# Autodesk Inventor assembly: Functioning elevator (frame 2)
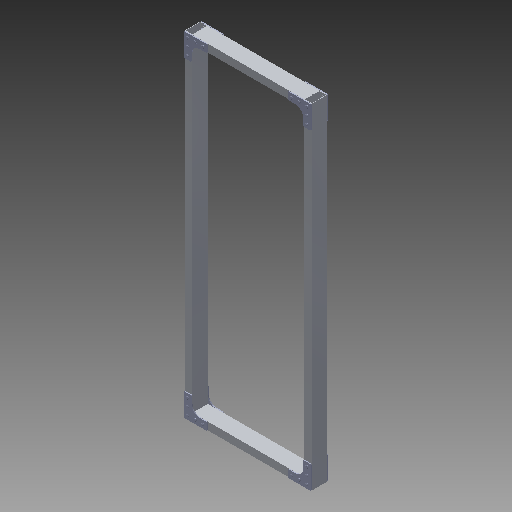
[picture p0: Inventor's stored thumbnail of the model, 512x512]
Saved by Autodesk Inventor 2019 (Build 230136000, 136)
## iProperties
Created: 2019-01-19
Part Number: Functioning elevator (frame 2)
Document SubType Name: Assembly
Designer: josh
Mass: 2087.98 g
Surface Area: 9404.6 cm^2
Volume: 773.327 cm^3
Density: 2.7 g/cm^3
Author: josh
## Documents named in this file (4)
- D:\Synthesis Robots\Epsilon\Epsilon elavator lift\Functioning elevator (frame 2).iam
- D:\Synthesis Robots\Epsilon\Epsilon elavator lift\Functioning elevator parts\Example Fixed Tube.ipt
- D:\Synthesis Robots\Epsilon\Epsilon elavator lift\Functioning elevator parts\am-3860 90 Gusset with Rivets.iam
- D:\Synthesis Robots\Epsilon\Epsilon elavator lift\Functioning elevator parts\Example Cross Frame Tube - Copy.ipt
## Components (12 placed, 3 different names)
1. Example Fixed Tube:1 — Mate:12, Flush:24, Mate:16, Flush:29, Flush:30, Flush:31, Mate:20, Flush:32
2. Example Fixed Tube:2 — Flush:22, Flush:23, Mate:14, Mate:15, Mate:17, Mate:18
3. am-3860 90 Gusset with Rivets:1 [sub-assembly] — Flush:22
4. am-3860 90 Gusset with Rivets:2 [sub-assembly] — Flush:23, Flush:25, Mate:13, Mate:14
5. am-3860 90 Gusset with Rivets:3 [sub-assembly] — Mate:11, Mate:12, Flush:24
6. am-3860 90 Gusset with Rivets:4 [sub-assembly] — Mate:10, Flush:32, Flush:33
7. am-3860 90 Gusset with Rivets:5 [sub-assembly] — Mate:18, Mate:19, Flush:27
8. am-3860 90 Gusset with Rivets:6 [sub-assembly] — Flush:26
9. am-3860 90 Gusset with Rivets:7 [sub-assembly] — Flush:28, Flush:29
10. am-3860 90 Gusset with Rivets:8 [sub-assembly] — Flush:30, Flush:31, Mate:20
11. Example Cross Frame Tube - Copy:1 — Mate:17, Mate:19, Flush:26, Flush:27, Flush:28
12. Example Cross Frame Tube - Copy:2 — Mate:10, Mate:11, Flush:25, Mate:13, Mate:15, Mate:16, Flush:33
## Relationships (38: Flush 24, Mate 14)
- [Flush]: Example Fixed Tube:2 ↔ am-3860 90 Gusset with Rivets:6
- [Flush]: Example Fixed Tube:2 ↔ am-3860 90 Gusset with Rivets:5
- [Mate]: Example Fixed Tube:2 ↔ am-3860 90 Gusset with Rivets:6
- [Flush]: Example Fixed Tube:2 ↔ am-3860 90 Gusset with Rivets:6
- [Flush]: Example Fixed Tube:2 ↔ am-3860 90 Gusset with Rivets:5
- [Flush]: Example Fixed Tube:2 ↔ am-3860 90 Gusset with Rivets:5
- [Mate]: Example Fixed Tube:1 ↔ am-3860 90 Gusset with Rivets:7
- [Flush]: Example Fixed Tube:1 ↔ am-3860 90 Gusset with Rivets:7
- [Flush]: Example Fixed Tube:1 ↔ am-3860 90 Gusset with Rivets:8
- [Flush]: Example Fixed Tube:2 ↔ am-3860 90 Gusset with Rivets:1
- [Mate]: Example Fixed Tube:2 ↔ am-3860 90 Gusset with Rivets:1
- [Flush]: Example Fixed Tube:2 ↔ am-3860 90 Gusset with Rivets:2
- [Flush]: Example Fixed Tube:1 ↔ am-3860 90 Gusset with Rivets:3
- [Flush]: Example Fixed Tube:1 ↔ am-3860 90 Gusset with Rivets:4
- [Flush]: Example Fixed Tube:1 ↔ am-3860 90 Gusset with Rivets:3
- Flush:22: Example Fixed Tube:2 ↔ am-3860 90 Gusset with Rivets:1
- Flush:23: Example Fixed Tube:2 ↔ am-3860 90 Gusset with Rivets:2
- Mate:10: am-3860 90 Gusset with Rivets:4 ↔ Example Cross Frame Tube - Copy:2
- Mate:11: am-3860 90 Gusset with Rivets:3 ↔ Example Cross Frame Tube - Copy:2
- Mate:12: Example Fixed Tube:1 ↔ am-3860 90 Gusset with Rivets:3
- Flush:24: Example Fixed Tube:1 ↔ am-3860 90 Gusset with Rivets:3
- Flush:25: am-3860 90 Gusset with Rivets:2 ↔ Example Cross Frame Tube - Copy:2
- Mate:13: am-3860 90 Gusset with Rivets:2 ↔ Example Cross Frame Tube - Copy:2
- Mate:14: Example Fixed Tube:2 ↔ am-3860 90 Gusset with Rivets:2
- Mate:15: Example Fixed Tube:2 ↔ Example Cross Frame Tube - Copy:2
- Mate:16: Example Fixed Tube:1 ↔ Example Cross Frame Tube - Copy:2
- Mate:17: Example Fixed Tube:2 ↔ Example Cross Frame Tube - Copy:1
- Mate:18: Example Fixed Tube:2 ↔ am-3860 90 Gusset with Rivets:5
- Mate:19: am-3860 90 Gusset with Rivets:5 ↔ Example Cross Frame Tube - Copy:1
- Flush:26: am-3860 90 Gusset with Rivets:6 ↔ Example Cross Frame Tube - Copy:1
- Flush:27: am-3860 90 Gusset with Rivets:5 ↔ Example Cross Frame Tube - Copy:1
- Flush:28: am-3860 90 Gusset with Rivets:7 ↔ Example Cross Frame Tube - Copy:1
- Flush:29: Example Fixed Tube:1 ↔ am-3860 90 Gusset with Rivets:7
- Flush:30: Example Fixed Tube:1 ↔ am-3860 90 Gusset with Rivets:8
- Flush:31: Example Fixed Tube:1 ↔ am-3860 90 Gusset with Rivets:8
- Mate:20: Example Fixed Tube:1 ↔ am-3860 90 Gusset with Rivets:8
- Flush:32: Example Fixed Tube:1 ↔ am-3860 90 Gusset with Rivets:4
- Flush:33: am-3860 90 Gusset with Rivets:4 ↔ Example Cross Frame Tube - Copy:2
## Named parameters: d1_d2 = 0 mm, d2_d3 = 0 mm, d5_d6 = 0 mm, d6_d7 = 0 mm, d7_d8 = 0 mm, d8_d9 = 0 mm, d12_d13 = 0 mm, d13_d14 = 0 mm, d16_d17 = 0 mm, d19_d20 = 0 mm, d21_d22 = 0 mm, d23_d24 = 0 mm, d28_d29 = 0 mm, d30_d31 = 0 mm, d33_d34 = 0 mm
